# Autodesk Inventor assembly: fabrication model end cap right
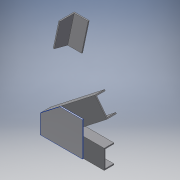
[picture p0: Inventor's stored thumbnail of the model, 180x180]
Saved by Autodesk Inventor 2016 (Build 200138000, 138)
## iProperties
Created: 2015-02-04
Part Number: fabrication model end cap right
Document SubType Name: Assembly
Designer: degan
Author: degan
## Documents named in this file (5)
- C:\Users\ddeboer\Desktop\hera-cad\support\endcaps-ChannelVersion\HERA_end_cap_right.iam
- C:\Users\ddeboer\Desktop\hera-cad\support\endcaps-ChannelVersion\angle channel.ipt
- C:\Users\ddeboer\Desktop\hera-cad\support\endcaps-ChannelVersion\ring support right.ipt
- C:\Users\ddeboer\Desktop\hera-cad\support\endcaps-ChannelVersion\Horizontal channel right.ipt
- C:\Users\ddeboer\Desktop\hera-cad\support\endcaps-ChannelVersion\side plate.ipt
## Components (4 placed, 4 different names)
1. side plate:1 — Mate:1, Flush:1, Mate:2, Flush:2
2. ring support right:1
3. angle channel:1 — Mate:1, Flush:1
4. Horizontal channel right:1 — Mate:2, Flush:2
## Relationships (4: Mate 2, Flush 2)
- Mate:1: side plate:1 ↔ angle channel:1
- Flush:1: side plate:1 ↔ angle channel:1
- Mate:2: side plate:1 ↔ Horizontal channel right:1
- Flush:2: side plate:1 ↔ Horizontal channel right:1
